# Autodesk Inventor assembly: x_axis
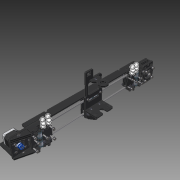
[picture p0: Inventor's stored thumbnail of the model, 180x180]
Saved by Autodesk Inventor 2014 (Build 180170000, 170)
## iProperties
Created: 2014-01-10
Part Number: x_axis
Document SubType Name: Assembly
Designer: buben
Author: buben
## Documents named in this file (9)
- C:\Users\buben\Documents\GitHub\bacon\inventor files\assemblies\x_axis.iam
- C:\Users\buben\Documents\GitHub\bacon\inventor files\assemblies\x_motor.iam
- C:\Users\buben\Documents\GitHub\bacon\inventor files\assemblies\x_iddler.iam
- C:\Users\buben\Documents\GitHub\bacon\inventor files\printer parts\x_axis_chain_holder.ipt
- C:\Users\buben\Documents\GitHub\bacon\inventor files\utils\x_axis_rod.ipt
- C:\Users\buben\Documents\GitHub\bacon\inventor files\assemblies\x_carryage.iam
- C:\Users\buben\Documents\GitHub\bacon\inventor files\utils\washer_m4.ipt
- C:\Users\buben\Documents\Inventor\Content Center Files\R2014\en-US\ISO 7040\ISO 7040 - M4.ipt
- C:\Users\buben\Documents\Inventor\Content Center Files\R2014\en-US\ISO 4762(2)\ISO 4762 - M4 x 30ISO.ipt
## Components (22 placed, 8 different names)
1. x_motor:1 [sub-assembly] — Mate:1, Mate:2, Mate:3, Flush:1, Flush:2, Tangent:1, Tangent:2, Tangent:3, Tangent:4, Tangent:5, Tangent:6, Mate:4, Mate:5, Mate:6, Mate:17, Mate:18, Mate:19, Mate:20
2. x_iddler:1 [sub-assembly] — Flush:1, Flush:2, Tangent:7, Mate:21, Mate:22, Mate:23, Mate:24
3. x_axis_chain_holder:1 — Mate:4, Mate:5, Mate:6, Mate:9, Mate:10, Mate:11, Mate:12, Mate:13, Mate:14, Mate:15, Mate:16
4. x_axis_rod:1 — Tangent:2, Tangent:4, Tangent:5, Tangent:7, Mate:7
5. x_axis_rod:2 — Tangent:1, Tangent:3, Tangent:6, Mate:8
6. x_carryage:1 [sub-assembly] — Mate:7, Mate:8
7. CSN 02 1702 B B 4,3:1 — Mate:21, Mate:23, Mate:29
8. CSN 02 1702 B B 4,3:2 — Mate:19, Mate:20, Mate:25
9. CSN 02 1702 B B 4,3:3 — Mate:22, Mate:24, Mate:31
10. CSN 02 1702 B B 4,3:4 — Mate:17, Mate:18, Mate:27
11. CSN 02 1702 B B 4,3:5 — Mate:12, Mate:13, Insert:4
12. CSN 02 1702 B B 4,3:6 — Mate:11, Mate:14, Insert:3
13. CSN 02 1702 B B 4,3:7 — Mate:10, Mate:15, Insert:2
14. CSN 02 1702 B B 4,3:8 — Mate:9, Mate:16, Insert:1
15. ISO 4762 M4 x 30:2 — Insert:1, Mate:28
16. ISO 4762 M4 x 30:1 — Insert:2, Mate:26
17. ISO 4762 M4 x 30:4 — Insert:3, Mate:32
18. ISO 4762 M4 x 30:3 — Insert:4, Mate:30
19. DIN EN ISO 7040 M4:1 — Mate:31, Mate:32
20. DIN EN ISO 7040 M4:2 — Mate:29, Mate:30
21. DIN EN ISO 7040 M4:3 — Mate:27, Mate:28
22. DIN EN ISO 7040 M4:4 — Mate:25, Mate:26
## Relationships (45: Mate 32, Tangent 7, Insert 4, Flush 2)
- Mate:1: x_motor:1
- Mate:2: x_motor:1
- Mate:3: x_motor:1
- Flush:1: x_motor:1 ↔ x_iddler:1
- Flush:2: x_motor:1 ↔ x_iddler:1
- Tangent:1: x_motor:1 ↔ x_axis_rod:2
- Tangent:2: x_motor:1 ↔ x_axis_rod:1
- Tangent:3: x_motor:1 ↔ x_axis_rod:2
- Tangent:4: x_motor:1 ↔ x_axis_rod:1
- Tangent:5: x_motor:1 ↔ x_axis_rod:1
- Tangent:6: x_motor:1 ↔ x_axis_rod:2
- Tangent:7: x_iddler:1 ↔ x_axis_rod:1
- Mate:4: x_motor:1 ↔ x_axis_chain_holder:1
- Mate:5: x_motor:1 ↔ x_axis_chain_holder:1
- Mate:6: x_motor:1 ↔ x_axis_chain_holder:1
- Mate:7: x_axis_rod:1 ↔ x_carryage:1
- Mate:8: x_axis_rod:2 ↔ x_carryage:1
- Mate:9: x_axis_chain_holder:1 ↔ CSN 02 1702 B B 4,3:8
- Mate:10: x_axis_chain_holder:1 ↔ CSN 02 1702 B B 4,3:7
- Mate:11: x_axis_chain_holder:1 ↔ CSN 02 1702 B B 4,3:6
- Mate:12: x_axis_chain_holder:1 ↔ CSN 02 1702 B B 4,3:5
- Mate:13: x_axis_chain_holder:1 ↔ CSN 02 1702 B B 4,3:5
- Mate:14: x_axis_chain_holder:1 ↔ CSN 02 1702 B B 4,3:6
- Mate:15: x_axis_chain_holder:1 ↔ CSN 02 1702 B B 4,3:7
- Mate:16: x_axis_chain_holder:1 ↔ CSN 02 1702 B B 4,3:8
- Mate:17: x_motor:1 ↔ CSN 02 1702 B B 4,3:4
- Mate:18: x_motor:1 ↔ CSN 02 1702 B B 4,3:4
- Mate:19: x_motor:1 ↔ CSN 02 1702 B B 4,3:2
- Mate:20: x_motor:1 ↔ CSN 02 1702 B B 4,3:2
- Mate:21: x_iddler:1 ↔ CSN 02 1702 B B 4,3:1
- Mate:22: x_iddler:1 ↔ CSN 02 1702 B B 4,3:3
- Mate:23: x_iddler:1 ↔ CSN 02 1702 B B 4,3:1
- Mate:24: x_iddler:1 ↔ CSN 02 1702 B B 4,3:3
- Insert:1: CSN 02 1702 B B 4,3:8 ↔ ISO 4762 M4 x 30:2
- Insert:2: CSN 02 1702 B B 4,3:7 ↔ ISO 4762 M4 x 30:1
- Insert:3: CSN 02 1702 B B 4,3:6 ↔ ISO 4762 M4 x 30:4
- Insert:4: CSN 02 1702 B B 4,3:5 ↔ ISO 4762 M4 x 30:3
- Mate:25: CSN 02 1702 B B 4,3:2 ↔ DIN EN ISO 7040 M4:4
- Mate:26: ISO 4762 M4 x 30:1 ↔ DIN EN ISO 7040 M4:4
- Mate:27: CSN 02 1702 B B 4,3:4 ↔ DIN EN ISO 7040 M4:3
- Mate:28: ISO 4762 M4 x 30:2 ↔ DIN EN ISO 7040 M4:3
- Mate:29: CSN 02 1702 B B 4,3:1 ↔ DIN EN ISO 7040 M4:2
- Mate:30: ISO 4762 M4 x 30:3 ↔ DIN EN ISO 7040 M4:2
- Mate:31: CSN 02 1702 B B 4,3:3 ↔ DIN EN ISO 7040 M4:1
- Mate:32: ISO 4762 M4 x 30:4 ↔ DIN EN ISO 7040 M4:1
